# Autodesk Inventor assembly: main
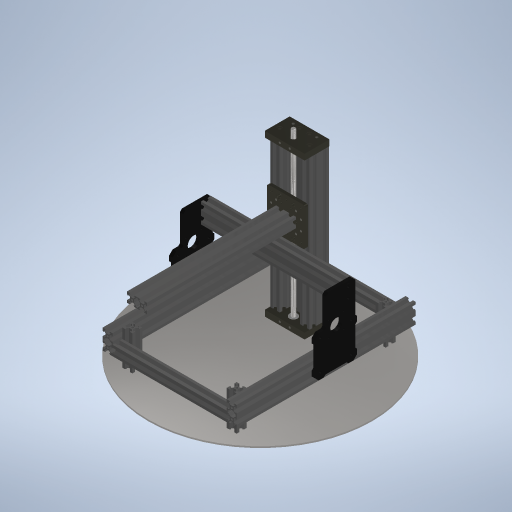
[picture p0: Inventor's stored thumbnail of the model, 512x512]
Saved by Autodesk Inventor 2024.3 (Build 283343000, 343)
## iProperties
Created: 2024-08-26
Part Number: main
Document SubType Name: Assembly
Designer: Admin
Author: Admin
## Documents named in this file (6)
- C:\Users\migue\Documents\GitHub\RobotCartesiano\DiseñoBrazo\Assemblies\main.iam
- C:\Users\migue\Documents\GitHub\RobotCartesiano\DiseñoBrazo\Assemblies\AxisX.iam
- C:\Users\migue\Documents\GitHub\RobotCartesiano\DiseñoBrazo\AuxiliarPieces\FestinoRobot\AluminumBase.ipt
- C:\Users\migue\Documents\GitHub\RobotCartesiano\DiseñoBrazo\Assemblies\MovingPlate.iam
- C:\Users\migue\Documents\GitHub\RobotCartesiano\DiseñoBrazo\Assemblies\StuctureZ.iam
- C:\Users\migue\Documents\GitHub\RobotCartesiano\DiseñoBrazo\Assemblies\AxisY.iam
## Components (5 placed, 5 different names)
1. AluminumBase:1 — Mate:1
2. AxisX:1 [sub-assembly] — Mate:1
3. MovingPlate:1 [sub-assembly] — Mate:2
4. StuctureZ:1 [sub-assembly] — Mate:2
5. AxisY:1 [sub-assembly]
## Relationships (2: Mate 2)
- Mate:1: AluminumBase:1 ↔ AxisX:1
- Mate:2: MovingPlate:1 ↔ StuctureZ:1
